# Autodesk Inventor assembly: PingPong
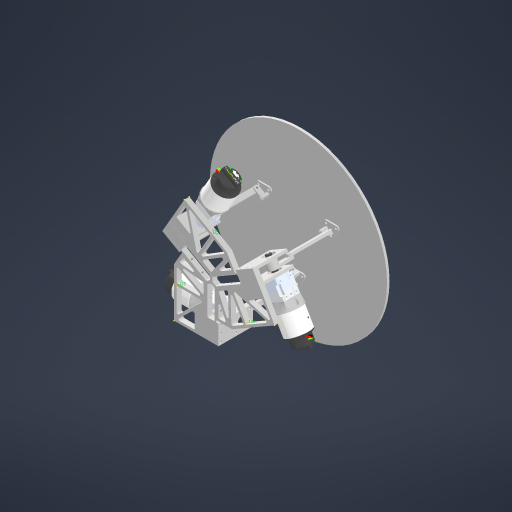
[picture p0: Inventor's stored thumbnail of the model, 512x512]
Saved by Autodesk Inventor 2023 (Build 270158000, 158)
## iProperties
Created: 2022-05-02
Part Number: PingPong
Document SubType Name: Assembly
Designer: FizzyApple12
Author: FizzyApple12
## Documents named in this file (3)
- C:\Users\FizzyApple12\Desktop\Ping Pong Robot\PingPong.iam
- C:\Users\FizzyApple12\Desktop\Ping Pong Robot\Third.iam
- C:\Users\FizzyApple12\Desktop\Ping Pong Robot\Table.ipt
## Components (4 placed, 2 different names)
1. Third:1 [sub-assembly] — Flush:1, Mate:2, Mate:3
2. Third:2 [sub-assembly] — Flush:1, Flush:2, Mate:1, Mate:2
3. Third:3 [sub-assembly] — Flush:2, Mate:1, Mate:3, Mate:4, Mate:5, Mate:6
4. Table:1 — Mate:4, Mate:5, Mate:6
## Relationships (8: Mate 6, Flush 2)
- Flush:1: Third:1 ↔ Third:2
- Flush:2: Third:2 ↔ Third:3
- Mate:1: Third:2 ↔ Third:3
- Mate:2: Third:1 ↔ Third:2
- Mate:3: Third:1 ↔ Third:3
- Mate:4: Third:3 ↔ Table:1
- Mate:5: Third:3 ↔ Table:1
- Mate:6: Third:3 ↔ Table:1
